# Autodesk Inventor assembly: Battery_holder
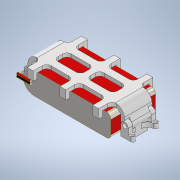
[picture p0: Inventor's stored thumbnail of the model, 180x180]
Saved by Autodesk Inventor 2022 (Build 260153000, 153)
## iProperties
Created: 2023-01-30
Part Number: Battery_holder
Document SubType Name: Assembly
Designer: scott
Author: scott
## Documents named in this file (4)
- C:\Users\scott\OneDrive\Documents\Cat project\Git_repository\Flinders_OpenCat\CAD components\Battery_holder.iam
- C:\Users\scott\OneDrive\Documents\Cat project\Git_repository\Flinders_OpenCat\CAD components\Battery_temp.ipt
- C:\Users\scott\OneDrive\Documents\Cat project\Git_repository\Flinders_OpenCat\CAD components\Battery_short_holder.ipt
- C:\Users\scott\OneDrive\Documents\Cat project\Git_repository\Flinders_OpenCat\CAD components\Battery_holder.ipt
## Components (4 placed, 3 different names)
1. Battery_short_holder:1 — Mate:1, Mate:2, Flush:1
2. Battery_short_holder:2 — Mate:3, Mate:4, Flush:1, Mate:6
3. Battery_holder:1 — Mate:1, Mate:2, Mate:3, Mate:4, Mate:5, Mate:7
4. Battery_temp:1 — Mate:5, Mate:6, Mate:7
## Relationships (8: Mate 7, Flush 1)
- Mate:1: Battery_short_holder:1 ↔ Battery_holder:1
- Mate:2: Battery_short_holder:1 ↔ Battery_holder:1
- Mate:3: Battery_short_holder:2 ↔ Battery_holder:1
- Mate:4: Battery_short_holder:2 ↔ Battery_holder:1
- Flush:1: Battery_short_holder:1 ↔ Battery_short_holder:2
- Mate:5: Battery_holder:1 ↔ Battery_temp:1
- Mate:6 (7.5 mm): Battery_short_holder:2 ↔ Battery_temp:1
- Mate:7 (0.75 mm): Battery_holder:1 ↔ Battery_temp:1
